# Autodesk Inventor assembly: BoronHead
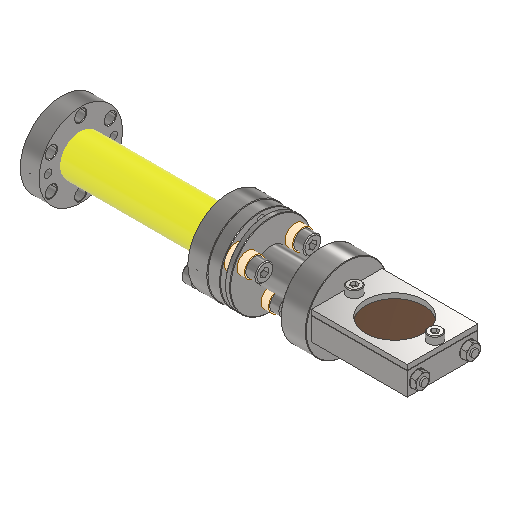
[picture p0: Inventor's stored thumbnail of the model, 512x512]
Saved by Autodesk Inventor 2026.2 (Build 302298000, 298)
## iProperties
Created: 2025-06-19
Part Number: BoronHead
Document SubType Name: Assembly
Designer: kuzmin
Author: kuzmin
## Documents named in this file (13)
- D:\repos\PIHTI\BoronProbe\BoronHead.iam
- D:\repos\PIHTI\BoronProbe\HayashiProbeHead.ipt
- D:\repos\PIHTI\ContentCenter\Fastners\M4x10-SHCS.ipt
- D:\repos\PIHTI\BoronProbe\Shaft.ipt
- D:\repos\PIHTI\ContentCenter\Ceramics\ceramic_bushing_M4.ipt
- D:\repos\PIHTI\ContentCenter\Ceramics\ceramic_washer_M4.ipt
- D:\repos\PIHTI\PALP\CF34-nipples-for-PALP\ICF34_70mmNipple.iam
- D:\repos\PIHTI\BoronProbe\flange-adapter.ipt
- D:\repos\PIHTI\BoronProbe\HayashiProbeHead_sub.ipt
- D:\repos\PIHTI\BoronProbe\HayashiProbeHead_up.ipt
- D:\repos\PIHTI\BoronProbe\substrate.ipt
- D:\repos\PIHTI\ContentCenter\Fastners\M3x10-SHCS.ipt
- D:\repos\PIHTI\ContentCenter\Fastners\M3-nut.ipt
## Components (23 placed, 12 different names)
1. HayashiProbeHead:1 — リジッド:4, リジッド:5, リジッド:6, 回転:1, 回転:2, リジッド:7, リジッド:8, リジッド:9, メイト:1, メイト:2, メイト:5
2. Shaft:1 — リジッド:5, メイト:7, 挿入:4
3. Shaft:2 — リジッド:4, メイト:6, 挿入:3
4. ceramic_bushing_M4:1 — リジッド:6, 回転:5
5. ceramic_bushing_M4:2 — 回転:1, 回転:4
6. ceramic_bushing_M4:3 — 回転:2, 回転:3
7. ceramic_washer_M4:1 — リジッド:7
8. ceramic_washer_M4:2 — リジッド:8
9. ceramic_washer_M4:3 — リジッド:9, メイト:4
10. ICF34_70mmNipple:1 [sub-assembly] — メイト:1, リジッド:10, リジッド:11, 回転:6
11. flange-adapter:1 — メイト:2, メイト:3, メイト:4, リジッド:10
12. AS 1420 - Metric M4 x 10:4 — リジッド:11
13. AS 1420 - Metric M4 x 10:5 — 回転:6
14. HayashiProbeHead_sub:1 — メイト:5, メイト:6, メイト:7, メイト:8, メイト:9, メイト:11, メイト:12
15. HayashiProbeHead_up:1 — メイト:10, メイト:11, メイト:12, 挿入:1, 挿入:2
16. substrate:1 — メイト:8, メイト:9, メイト:10
17. JIS B 1176 - Metric M3 x 10:1 — 挿入:2
18. JIS B 1176 - Metric M3 x 10:2 — 挿入:1
19. JIS B 1181 Style 1 - Metric A M3:1 — 挿入:3
20. JIS B 1181 Style 1 - Metric A M3:2 — 挿入:4
21. AS 1420 - Metric M4 x 10:1 — 回転:4
22. AS 1420 - Metric M4 x 10:2 — 回転:5, メイト:3
23. AS 1420 - Metric M4 x 10:3 — 回転:3
## Relationships (30: Mate 12, WeldJoint 8, RevoluteJoint 6, Insert 4)
- リジッド:4 [WeldJoint]: HayashiProbeHead:1 ↔ Shaft:2
- リジッド:5 [WeldJoint]: HayashiProbeHead:1 ↔ Shaft:1
- リジッド:6 [WeldJoint]: HayashiProbeHead:1 ↔ ceramic_bushing_M4:1
- 回転:1 [RevoluteJoint]: HayashiProbeHead:1 ↔ ceramic_bushing_M4:2
- 回転:2 [RevoluteJoint]: HayashiProbeHead:1 ↔ ceramic_bushing_M4:3
- 回転:3 [RevoluteJoint]: ceramic_bushing_M4:3 ↔ AS 1420 - Metric M4 x 10:3
- 回転:4 [RevoluteJoint]: ceramic_bushing_M4:2 ↔ AS 1420 - Metric M4 x 10:1
- 回転:5 [RevoluteJoint]: ceramic_bushing_M4:1 ↔ AS 1420 - Metric M4 x 10:2
- リジッド:7 [WeldJoint]: HayashiProbeHead:1 ↔ ceramic_washer_M4:1
- リジッド:8 [WeldJoint]: HayashiProbeHead:1 ↔ ceramic_washer_M4:2
- リジッド:9 [WeldJoint]: HayashiProbeHead:1 ↔ ceramic_washer_M4:3
- メイト:1 [Mate]: HayashiProbeHead:1 ↔ ICF34_70mmNipple:1
- メイト:2 [Mate]: HayashiProbeHead:1 ↔ flange-adapter:1
- メイト:3 [Mate]: flange-adapter:1 ↔ AS 1420 - Metric M4 x 10:2
- メイト:4 [Mate]: ceramic_washer_M4:3 ↔ flange-adapter:1
- リジッド:10 [WeldJoint]: ICF34_70mmNipple:1 ↔ flange-adapter:1
- リジッド:11 [WeldJoint]: ICF34_70mmNipple:1 ↔ AS 1420 - Metric M4 x 10:4
- 回転:6 [RevoluteJoint]: ICF34_70mmNipple:1 ↔ AS 1420 - Metric M4 x 10:5
- メイト:5 [Mate]: HayashiProbeHead:1 ↔ HayashiProbeHead_sub:1
- メイト:6 [Mate]: Shaft:2 ↔ HayashiProbeHead_sub:1
- メイト:7 [Mate]: Shaft:1 ↔ HayashiProbeHead_sub:1
- メイト:8 [Mate]: HayashiProbeHead_sub:1 ↔ substrate:1
- メイト:9 [Mate]: HayashiProbeHead_sub:1 ↔ substrate:1
- メイト:10 [Mate]: HayashiProbeHead_up:1 ↔ substrate:1
- メイト:11 [Mate]: HayashiProbeHead_sub:1 ↔ HayashiProbeHead_up:1
- メイト:12 [Mate]: HayashiProbeHead_sub:1 ↔ HayashiProbeHead_up:1
- 挿入:1 [Insert]: HayashiProbeHead_up:1 ↔ JIS B 1176 - Metric M3 x 10:2
- 挿入:2 [Insert]: HayashiProbeHead_up:1 ↔ JIS B 1176 - Metric M3 x 10:1
- 挿入:3 [Insert]: Shaft:2 ↔ JIS B 1181 Style 1 - Metric A M3:1
- 挿入:4 [Insert]: Shaft:1 ↔ JIS B 1181 Style 1 - Metric A M3:2
